# Autodesk Inventor assembly: Adjustable Elbow 1 Inch - Sax Angle
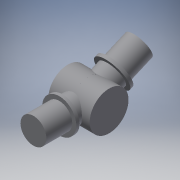
[picture p0: Inventor's stored thumbnail of the model, 180x180]
Saved by Autodesk Inventor 2018.2 (Build 222227000, 227)
## iProperties
Created: 2018-01-10
Part Number: Adjustable Elbow 1 Inch - Sax Angle
Document SubType Name: Assembly
Designer: owner
Author: owner
## Documents named in this file (2)
- Z:\The Pickle - 4 - Copy\Final Carts\Sax Cart\Adjustable Elbow 1 Inch - Sax Angle.iam
- Z:\The Pickle - 4 - Copy\Final Carts\Sax Cart\Adjustable Elbow\Adjustable elbow piece 1 inch.ipt
## Components (2 placed, 1 different names)
1. Adjustable elbow piece 1 inch:1 — Mate:1, Angle:1
2. Adjustable elbow piece 1 inch:2 — Mate:1, Angle:1
## Relationships (2: Mate 1, Angle 1)
- Mate:1: Adjustable elbow piece 1 inch:1 ↔ Adjustable elbow piece 1 inch:2
- Angle:1 (156.863 deg): Adjustable elbow piece 1 inch:1 ↔ Adjustable elbow piece 1 inch:2
